# Autodesk Inventor assembly: Cover
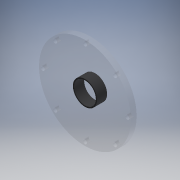
[picture p0: Inventor's stored thumbnail of the model, 180x180]
Saved by Autodesk Inventor 2017 (Build 210142000, 142)
## iProperties
Created: 2016-10-31
Part Number: Cover
Document SubType Name: Assembly
Designer: Andres
Author: Andres
## Documents named in this file (4)
- Z:\Documents\repositorios\BoreholeCamera\CAD_Probe\Enclosure\Assembly\Cover.iam
- \\Mac\Home\Documents\repositorios\BoreholeCamera\CAD_Probe\Enclosure\Parts\Cover.ipt
- \\Mac\Home\Documents\repositorios\BoreholeCamera\CAD_Probe\Enclosure\Parts\CoverPart1.ipt
- \\Mac\Home\Documents\repositorios\BoreholeCamera\CAD_Probe\Enclosure\Parts\CoverPart2.ipt
## Components (3 placed, 3 different names)
1. Cover:1 — Rigid:1
2. CoverPart1:1 — Rigid:1, Rigid:2
3. CoverPart2:1 — Rigid:2
## Relationships (2: WeldJoint 2)
- Rigid:1 [WeldJoint]: Cover:1 ↔ CoverPart1:1
- Rigid:2 [WeldJoint]: CoverPart1:1 ↔ CoverPart2:1
